# Autodesk Inventor assembly: КВ33.044.200 - Каретка оси Х
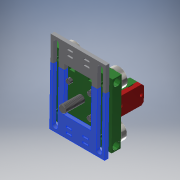
[picture p0: Inventor's stored thumbnail of the model, 180x180]
Saved by Autodesk Inventor 2019 (Build 230136000, 136)
## iProperties
Created: 2019-07-16
Part Number: КВ33.044.200 - Каретка оси Х
Material: Типовые
Document SubType Name: Assembly
Designer: Петров Иван
Author: Петров Иван
## Documents named in this file (8)
- E:\IVAN\Kvantoriada2019\optimal_gripper\hardware\КВ33.044.200 - Каретка оси Z.iam
- E:\IVAN\Kvantoriada2019\optimal_gripper\hardware\КВ33.044.201 - Щека каретки Z.ipt
- E:\IVAN\Kvantoriada2019\optimal_gripper\hardware\Стандартные изделия\Подшипник 626Z.ipt
- E:\IVAN\Kvantoriada2019\optimal_gripper\hardware\Стандартные изделия\Подшипник 624Z.ipt
- E:\IVAN\Kvantoriada2019\optimal_gripper\hardware\Стандартные изделия\Винт М8х25 с потайной головкой.ipt
- E:\IVAN\Kvantoriada2019\optimal_gripper\hardware\Стандартные изделия\Винт М5х10 с потайной головкой.ipt
- E:\IVAN\Kvantoriada2019\optimal_gripper\hardware\КВ33.044.203 - Прижим ремня каретки Z.ipt
- E:\IVAN\Kvantoriada2019\optimal_gripper\hardware\КВ33.044.204 - Держатель ремня.ipt
## Components (17 placed, 7 different names)
1. КВ33.044.201 - Щека каретки Z:1 — Совмещение:1, Совмещение:2, Совмещение:3, Совмещение:4, Совмещение:5, Совмещение:6, Совмещение:7, Совмещение:8, Совмещение:9, Совмещение:10, Совмещение:11, Совмещение:12, Совмещение:13, Совмещение:14, Совмещение:15, Совмещение:16, Совмещение:20, Заподлицо:1, Совмещение:21, Совмещение:22, Совмещение:23, Совмещение:24, Заподлицо:2, Заподлицо:3, Заподлицо:4, Заподлицо:5, Совмещение:25, Совмещение:26, Совмещение:27, Касательность:1, Касательность:2, Совмещение:28, Касательность:3, Касательность:4, Совмещение:29
2. Подшипник 626Z:1 — Совмещение:1, Совмещение:8
3. Подшипник 626Z:2 — Совмещение:2, Совмещение:5
4. Подшипник 626Z:3 — Совмещение:3, Совмещение:7
5. Подшипник 626Z:4 — Совмещение:4, Совмещение:6
6. Подшипник 624Z:1 — Совмещение:9, Совмещение:10
7. Подшипник 624Z:2 — Совмещение:13, Совмещение:14
8. Подшипник 624Z:3 — Совмещение:11, Совмещение:12
9. Подшипник 624Z:4 — Совмещение:15, Совмещение:16
10. Винт М8х25 с потайной головкой:1 — Совмещение:20, Заподлицо:1
11. Винт М5х10 с потайной головкой:1 — Совмещение:22, Заподлицо:2
12. Винт М5х10 с потайной головкой:2 — Совмещение:24, Заподлицо:3
13. Винт М5х10 с потайной головкой:3 — Совмещение:21, Заподлицо:5
14. Винт М5х10 с потайной головкой:4 — Совмещение:23, Заподлицо:4
15. КВ33.044.203 - Прижим ремня каретки Z:1 — Совмещение:25, Совмещение:26, Совмещение:27
16. КВ33.044.204 - Держатель ремня:1 — Касательность:3, Касательность:4, Совмещение:29
17. КВ33.044.204 - Держатель ремня:2 — Касательность:1, Касательность:2, Совмещение:28
## Relationships (35: Mate 26, Flush 5, Tangent 4)
- Совмещение:1 [Mate]: КВ33.044.201 - Щека каретки Z:1 ↔ Подшипник 626Z:1
- Совмещение:2 [Mate]: КВ33.044.201 - Щека каретки Z:1 ↔ Подшипник 626Z:2
- Совмещение:3 [Mate]: КВ33.044.201 - Щека каретки Z:1 ↔ Подшипник 626Z:3
- Совмещение:4 [Mate]: КВ33.044.201 - Щека каретки Z:1 ↔ Подшипник 626Z:4
- Совмещение:5 [Mate] (1 mm): КВ33.044.201 - Щека каретки Z:1 ↔ Подшипник 626Z:2
- Совмещение:6 [Mate] (1 mm): КВ33.044.201 - Щека каретки Z:1 ↔ Подшипник 626Z:4
- Совмещение:7 [Mate] (1 mm): КВ33.044.201 - Щека каретки Z:1 ↔ Подшипник 626Z:3
- Совмещение:8 [Mate] (1 mm): КВ33.044.201 - Щека каретки Z:1 ↔ Подшипник 626Z:1
- Совмещение:9 [Mate]: КВ33.044.201 - Щека каретки Z:1 ↔ Подшипник 624Z:1
- Совмещение:10 [Mate] (0.5 mm): КВ33.044.201 - Щека каретки Z:1 ↔ Подшипник 624Z:1
- Совмещение:11 [Mate]: КВ33.044.201 - Щека каретки Z:1 ↔ Подшипник 624Z:3
- Совмещение:12 [Mate] (0.5 mm): КВ33.044.201 - Щека каретки Z:1 ↔ Подшипник 624Z:3
- Совмещение:13 [Mate]: КВ33.044.201 - Щека каретки Z:1 ↔ Подшипник 624Z:2
- Совмещение:14 [Mate] (0.5 mm): КВ33.044.201 - Щека каретки Z:1 ↔ Подшипник 624Z:2
- Совмещение:15 [Mate]: КВ33.044.201 - Щека каретки Z:1 ↔ Подшипник 624Z:4
- Совмещение:16 [Mate] (0.5 mm): КВ33.044.201 - Щека каретки Z:1 ↔ Подшипник 624Z:4
- Совмещение:20 [Mate]: КВ33.044.201 - Щека каретки Z:1 ↔ Винт М8х25 с потайной головкой:1
- Заподлицо:1 [Flush] (2 mm): КВ33.044.201 - Щека каретки Z:1 ↔ Винт М8х25 с потайной головкой:1
- Совмещение:21 [Mate]: КВ33.044.201 - Щека каретки Z:1 ↔ Винт М5х10 с потайной головкой:3
- Совмещение:22 [Mate]: КВ33.044.201 - Щека каретки Z:1 ↔ Винт М5х10 с потайной головкой:1
- Совмещение:23 [Mate]: КВ33.044.201 - Щека каретки Z:1 ↔ Винт М5х10 с потайной головкой:4
- Совмещение:24 [Mate]: КВ33.044.201 - Щека каретки Z:1 ↔ Винт М5х10 с потайной головкой:2
- Заподлицо:2 [Flush] (1 mm): КВ33.044.201 - Щека каретки Z:1 ↔ Винт М5х10 с потайной головкой:1
- Заподлицо:3 [Flush] (1 mm): КВ33.044.201 - Щека каретки Z:1 ↔ Винт М5х10 с потайной головкой:2
- Заподлицо:4 [Flush] (1 mm): КВ33.044.201 - Щека каретки Z:1 ↔ Винт М5х10 с потайной головкой:4
- Заподлицо:5 [Flush] (1 mm): КВ33.044.201 - Щека каретки Z:1 ↔ Винт М5х10 с потайной головкой:3
- Совмещение:25 [Mate]: КВ33.044.201 - Щека каретки Z:1 ↔ КВ33.044.203 - Прижим ремня каретки Z:1
- Совмещение:26 [Mate]: КВ33.044.201 - Щека каретки Z:1 ↔ КВ33.044.203 - Прижим ремня каретки Z:1
- Совмещение:27 [Mate]: КВ33.044.201 - Щека каретки Z:1 ↔ КВ33.044.203 - Прижим ремня каретки Z:1
- Касательность:1 [Tangent]: КВ33.044.201 - Щека каретки Z:1 ↔ КВ33.044.204 - Держатель ремня:2
- Касательность:2 [Tangent]: КВ33.044.201 - Щека каретки Z:1 ↔ КВ33.044.204 - Держатель ремня:2
- Совмещение:28 [Mate]: КВ33.044.201 - Щека каретки Z:1 ↔ КВ33.044.204 - Держатель ремня:2
- Касательность:3 [Tangent]: КВ33.044.201 - Щека каретки Z:1 ↔ КВ33.044.204 - Держатель ремня:1
- Касательность:4 [Tangent]: КВ33.044.201 - Щека каретки Z:1 ↔ КВ33.044.204 - Держатель ремня:1
- Совмещение:29 [Mate]: КВ33.044.201 - Щека каретки Z:1 ↔ КВ33.044.204 - Держатель ремня:1
